# Autodesk Inventor assembly: mini engine 101
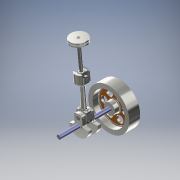
[picture p0: Inventor's stored thumbnail of the model, 180x180]
Saved by Autodesk Inventor 2017 (Build 210142000, 142)
## iProperties
Created: 2018-11-17
Part Number: mini engine 101
Document SubType Name: Assembly
Designer: User
Author: User
## Documents named in this file (12)
- C:\Users\User\Documents\engine\Good copy engine Sahil\mini engine 101.iam
- C:\Users\User\Documents\engine\Good copy engine Sahil\reverse gear fly wheel.ipt
- C:\Users\User\Documents\engine\Good copy engine Sahil\reverse gear crankshaft outer rod.ipt
- C:\Users\User\Documents\engine\Good copy engine Sahil\reverse gear crankshaft counter weight 2.ipt
- C:\Users\User\Documents\engine\Good copy engine Sahil\reverse gear bearing keeper.ipt
- C:\Users\User\Documents\engine\Good copy engine Sahil\reverse gear connecting rod 1.ipt
- C:\Users\User\Documents\engine\Good copy engine Sahil\reverse gear crankshaft center rod.ipt
- C:\Users\User\Documents\engine\Good copy engine Sahil\reverse gear crank rod 1.ipt
- C:\Users\User\Documents\engine\Good copy engine Sahil\reverse gear crankrod pin 1.ipt
- C:\Users\User\Documents\engine\Good copy engine Sahil\reverse gear cross head 1.ipt
- C:\Users\User\Documents\engine\Good copy engine Sahil\reverse gear pistion rod.ipt
- C:\Users\User\Documents\engine\Good copy engine Sahil\reverse gear piston.ipt
## Components (14 placed, 11 different names)
1. reverse gear fly wheel:1 — Insert:1, Rotation:1, Rotation:2, Rotation:3, Rotation:4, Rotation:5, Rotation:8, Rotation/Translation:2, Rotation:9, Rotation:11, Rotation/Translation:3, Rotation:15
2. reverse gear crankshaft outer rod:1 — Insert:1, Insert:2, Rotation:2, Rotation/Translation:1, Rotation:7, Rotation:12
3. reverse gear crankshaft counter weight 2:1 — Insert:2, Insert:3, Rotation:1
4. reverse gear bearing keeper:1 — Mate:2, Flush:3, Flush:4
5. reverse gear connecting rod 1:1 — Mate:1, Flush:1, Flush:2, Insert:4, Mate:3, Flush:5, Flush:6, Rotation/Translation:2
6. reverse gear connecting rod 1:2 — Mate:1, Flush:1, Flush:2, Mate:2, Flush:3, Flush:4
7. reverse gear crankshaft center rod:1 — Insert:3, Insert:4, Insert:5, Rotation:3
8. reverse gear crankshaft counter weight 2:2 — Insert:5, Rotation:4, Insert:6, Rotation:6
9. reverse gear crankshaft outer rod:2 — Insert:6
10. reverse gear crank rod 1:1 — Mate:3, Flush:5, Flush:6, Rotation:5, Rotation/Translation:1, Rotation:6, Rotation:7, Rotation:8, Insert:7, Rotation:10, Rotation:13, Rotation:14, Rotation:16
11. reverse gear crankrod pin 1:1 — Insert:7, Insert:8, Rotation:17
12. reverse gear cross head 1:1 — Insert:8, Rotation:9, Rotation:10, Rotation:11, Rotation:12, Rotation:13, Rotation:14, Rotation/Translation:3, Rotation:15, Rotation:16, Rotation:17, Insert:9
13. reverse gear pistion rod:1 — Insert:9, Insert:10
14. reverse gear piston:1 — Insert:10
## Relationships (39: RelateRotation 17, Insert 10, Flush 6, Mate 3, RelateRotateTranslate 3)
- Insert:1: reverse gear fly wheel:1 ↔ reverse gear crankshaft outer rod:1
- Insert:2: reverse gear crankshaft outer rod:1 ↔ reverse gear crankshaft counter weight 2:1
- Mate:1: reverse gear connecting rod 1:1 ↔ reverse gear connecting rod 1:2
- Flush:1: reverse gear connecting rod 1:1 ↔ reverse gear connecting rod 1:2
- Flush:2: reverse gear connecting rod 1:1 ↔ reverse gear connecting rod 1:2
- Mate:2: reverse gear bearing keeper:1 ↔ reverse gear connecting rod 1:2
- Flush:3: reverse gear bearing keeper:1 ↔ reverse gear connecting rod 1:2
- Flush:4: reverse gear bearing keeper:1 ↔ reverse gear connecting rod 1:2
- Insert:3 (-8 mm): reverse gear crankshaft counter weight 2:1 ↔ reverse gear crankshaft center rod:1
- Insert:4 (-17 mm): reverse gear connecting rod 1:1 ↔ reverse gear crankshaft center rod:1
- Insert:5 (-7 mm): reverse gear crankshaft center rod:1 ↔ reverse gear crankshaft counter weight 2:2
- Rotation:1 [RelateRotation] (1 ul): reverse gear fly wheel:1 ↔ reverse gear crankshaft counter weight 2:1
- Rotation:2 [RelateRotation] (1 ul): reverse gear fly wheel:1 ↔ reverse gear crankshaft outer rod:1
- Rotation:3 [RelateRotation] (1 ul): reverse gear fly wheel:1 ↔ reverse gear crankshaft center rod:1
- Rotation:4 [RelateRotation] (1 ul): reverse gear fly wheel:1 ↔ reverse gear crankshaft counter weight 2:2
- Insert:6 (-5 mm): reverse gear crankshaft counter weight 2:2 ↔ reverse gear crankshaft outer rod:2
- Mate:3: reverse gear connecting rod 1:1 ↔ reverse gear crank rod 1:1
- Flush:5: reverse gear connecting rod 1:1 ↔ reverse gear crank rod 1:1
- Flush:6: reverse gear connecting rod 1:1 ↔ reverse gear crank rod 1:1
- Rotation:5 [RelateRotation] (1 ul): reverse gear fly wheel:1 ↔ reverse gear crank rod 1:1
- Rotation/Translation:1 [RelateRotateTranslate] (1 mm): reverse gear crankshaft outer rod:1 ↔ reverse gear crank rod 1:1
- Rotation:6 [RelateRotation] (1 ul): reverse gear crankshaft counter weight 2:2 ↔ reverse gear crank rod 1:1
- Rotation:7 [RelateRotation] (1 ul): reverse gear crankshaft outer rod:1 ↔ reverse gear crank rod 1:1
- Rotation:8 [RelateRotation] (1 ul): reverse gear fly wheel:1 ↔ reverse gear crank rod 1:1
- Rotation/Translation:2 [RelateRotateTranslate] (1 mm): reverse gear fly wheel:1 ↔ reverse gear connecting rod 1:1
- Insert:7 (-1 mm): reverse gear crank rod 1:1 ↔ reverse gear crankrod pin 1:1
- Insert:8 (4 mm): reverse gear crankrod pin 1:1 ↔ reverse gear cross head 1:1
- Rotation:9 [RelateRotation] (1 ul): reverse gear fly wheel:1 ↔ reverse gear cross head 1:1
- Rotation:10 [RelateRotation] (1 ul): reverse gear crank rod 1:1 ↔ reverse gear cross head 1:1
- Rotation:11 [RelateRotation] (1 ul): reverse gear fly wheel:1 ↔ reverse gear cross head 1:1
- Rotation:12 [RelateRotation] (1 ul): reverse gear crankshaft outer rod:1 ↔ reverse gear cross head 1:1
- Rotation:13 [RelateRotation] (1 ul): reverse gear crank rod 1:1 ↔ reverse gear cross head 1:1
- Rotation:14 [RelateRotation] (0.6 ul): reverse gear crank rod 1:1 ↔ reverse gear cross head 1:1
- Rotation/Translation:3 [RelateRotateTranslate] (1 mm): reverse gear fly wheel:1 ↔ reverse gear cross head 1:1
- Rotation:15 [RelateRotation] (0.293 ul): reverse gear fly wheel:1 ↔ reverse gear cross head 1:1
- Rotation:16 [RelateRotation] (1 ul): reverse gear crank rod 1:1 ↔ reverse gear cross head 1:1
- Rotation:17 [RelateRotation] (1 ul): reverse gear crankrod pin 1:1 ↔ reverse gear cross head 1:1
- Insert:9 (-8 mm): reverse gear cross head 1:1 ↔ reverse gear pistion rod:1
- Insert:10: reverse gear pistion rod:1 ↔ reverse gear piston:1
